# Autodesk Inventor assembly: Base2
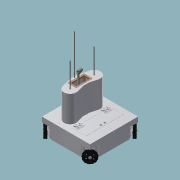
[picture p0: Inventor's stored thumbnail of the model, 180x180]
Saved by Autodesk Inventor 2017 SP1 (Build 210196100, 196)
## iProperties
Created: 2017-06-13
Part Number: Base2
Document SubType Name: Assembly
Designer: zallen
Author: zallen
## Documents named in this file (13)
- C:\Users\Zach\Documents\GitHub\tr1\src\Base\Base.iam
- C:\Users\Zach\Documents\GitHub\tr1\src\Base\Chassis\Chassis.iam
- C:\Users\Zach\Documents\GitHub\tr1\lib\Linear Actuator 300mm\LinearActuator300mm.iam
- C:\Users\Zach\Documents\GitHub\tr1\src\Base\Wheel Assembly\Wheel Assembly.iam
- C:\Users\Zach\Documents\GitHub\tr1\src\Base\Quick Shaft 10mm x 750mm.ipt
- C:\Users\Zach\Documents\GitHub\tr1\lib\ExpertPower EXP12180 Battery.ipt
- C:\Users\Zach\Documents\GitHub\tr1\src\Base\Battery Box\BatteryBox.iam
- C:\Users\Zach\Documents\GitHub\tr1\src\Base\Side Panel\Side Panel.iam
- C:\Users\Zach\Documents\GitHub\tr1\src\Base\Side Panel\Side Panel Front.iam
- C:\Users\Zach\Documents\GitHub\tr1\src\Base\Side Panel\Side Panel Back.iam
- C:\Users\Zach\Documents\GitHub\tr1\src\Base\Top Cover Assembly\Top Cover Assembly.iam
- C:\Users\Zach\Documents\GitHub\tr1\src\Base\Quick Shaft 10mm x 1000mm.ipt
- C:\Users\Zach\Documents\GitHub\tr1\src\Base\Riser Base Assembly - Solid\Riser Base Solid.iam
## Components (17 placed, 12 different names)
1. Chassis:1 [sub-assembly] — Mate:36, Mate:43, Mate:46, Mate:49, Mate:165, Flush:63, Mate:166, Flush:64, Mate:197, Mate:198, Mate:199, Flush:67, Mate:230, Mate:231, Mate:232, Mate:234, Mate:237, Mate:243, Mate:244, Mate:245, Mate:247, Mate:249, Mate:250, Mate:251, Mate:252, Mate:253, Mate:254, Mate:255, Mate:256
2. LinearActuator6inches:1 [sub-assembly] — Mate:197, Mate:198, Mate:199
3. Wheel Assembly:1 [sub-assembly] — Mate:36, Mate:251, Mate:252
4. Wheel Assembly:2 [sub-assembly] — Mate:43, Mate:249, Mate:250
5. Wheel Assembly:3 [sub-assembly] — Mate:46, Mate:255, Mate:256
6. Wheel Assembly:4 [sub-assembly] — Mate:49, Mate:253, Mate:254
7. Quick Shaft 10mm x 650mm:1 — Mate:223, Mate:227
8. Quick Shaft 10mm x 650mm:2 — Mate:224, Mate:226
9. Quick Shaft 10mm x 850mm:1 — Mate:222, Mate:228
10. ExpertPower EXP12180 Battery:1 — Mate:165, Mate:167
11. BatteryBox:1 [sub-assembly] — Flush:63, Mate:166, Flush:64, Mate:167
12. Side Panel:3 [sub-assembly] — Mate:237, Mate:238, Mate:239, Flush:69, Mate:241, Flush:70
13. Side Panel:4 [sub-assembly] — Mate:234, Mate:235, Mate:236
14. Side Panel Front:1 [sub-assembly] — Mate:232, Mate:233, Flush:68, Mate:236, Mate:239, Flush:69
15. Side Panel Back:1 [sub-assembly] — Mate:240, Mate:241, Flush:70, Flush:71
16. Top Cover Assembly:1 [sub-assembly] — Mate:233, Flush:68, Mate:235, Mate:238, Mate:240, Flush:71, Mate:246, Mate:247
17. Riser Base Solid:1 [sub-assembly] — Mate:222, Mate:223, Mate:224, Mate:226, Mate:227, Mate:228, Flush:67, Mate:230, Mate:231
## Relationships (48: Mate 41, Flush 7)
- Mate:36: Chassis:1 ↔ Wheel Assembly:1
- Mate:43: Chassis:1 ↔ Wheel Assembly:2
- Mate:46: Chassis:1 ↔ Wheel Assembly:3
- Mate:49: Chassis:1 ↔ Wheel Assembly:4
- Mate:165: Chassis:1 ↔ ExpertPower EXP12180 Battery:1
- Flush:63: Chassis:1 ↔ BatteryBox:1
- Mate:166: Chassis:1 ↔ BatteryBox:1
- Flush:64: Chassis:1 ↔ BatteryBox:1
- Mate:167: ExpertPower EXP12180 Battery:1 ↔ BatteryBox:1
- Mate:197: Chassis:1 ↔ LinearActuator6inches:1
- Mate:198: Chassis:1 ↔ LinearActuator6inches:1
- Mate:199: Chassis:1 ↔ LinearActuator6inches:1
- Mate:222: Quick Shaft 10mm x 850mm:1 ↔ Riser Base Solid:1
- Mate:223: Quick Shaft 10mm x 650mm:1 ↔ Riser Base Solid:1
- Mate:224: Quick Shaft 10mm x 650mm:2 ↔ Riser Base Solid:1
- Mate:226: Quick Shaft 10mm x 650mm:2 ↔ Riser Base Solid:1
- Mate:227: Quick Shaft 10mm x 650mm:1 ↔ Riser Base Solid:1
- Mate:228: Quick Shaft 10mm x 850mm:1 ↔ Riser Base Solid:1
- Flush:67: Chassis:1 ↔ Riser Base Solid:1
- Mate:230: Chassis:1 ↔ Riser Base Solid:1
- Mate:231: Chassis:1 ↔ Riser Base Solid:1
- Mate:232: Chassis:1 ↔ Side Panel Front:1
- Mate:233: Side Panel Front:1 ↔ Top Cover Assembly:1
- Flush:68: Side Panel Front:1 ↔ Top Cover Assembly:1
- Mate:234: Chassis:1 ↔ Side Panel:4
- Mate:235: Side Panel:4 ↔ Top Cover Assembly:1
- Mate:236: Side Panel:4 ↔ Side Panel Front:1
- Mate:237: Chassis:1 ↔ Side Panel:3
- Mate:238: Side Panel:3 ↔ Top Cover Assembly:1
- Mate:239: Side Panel:3 ↔ Side Panel Front:1
- Flush:69: Side Panel:3 ↔ Side Panel Front:1
- Mate:240: Side Panel Back:1 ↔ Top Cover Assembly:1
- Mate:241: Side Panel:3 ↔ Side Panel Back:1
- Flush:70: Side Panel:3 ↔ Side Panel Back:1
- Flush:71: Side Panel Back:1 ↔ Top Cover Assembly:1
- Mate:243: Chassis:1
- Mate:244: Chassis:1
- Mate:245 (-111.5 mm): Chassis:1
- Mate:246: Top Cover Assembly:1
- Mate:247: Chassis:1 ↔ Top Cover Assembly:1
- Mate:249: Chassis:1 ↔ Wheel Assembly:2
- Mate:250: Chassis:1 ↔ Wheel Assembly:2
- Mate:251: Chassis:1 ↔ Wheel Assembly:1
- Mate:252: Chassis:1 ↔ Wheel Assembly:1
- Mate:253: Chassis:1 ↔ Wheel Assembly:4
- Mate:254: Chassis:1 ↔ Wheel Assembly:4
- Mate:255: Chassis:1 ↔ Wheel Assembly:3
- Mate:256: Chassis:1 ↔ Wheel Assembly:3
